# Autodesk Inventor assembly: am-3479L+6+SR+Mecanum+Left
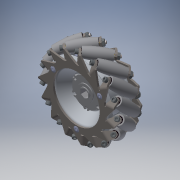
[picture p0: Inventor's stored thumbnail of the model, 180x180]
Saved by Autodesk Inventor 2016 SP2 (Build 200236200, 236)
## iProperties
Created: 2017-11-11
Part Number: am-3479L+6+SR+Mecanum+Left
Description: STEP AP214
Document SubType Name: Assembly
Designer: CAD
Sending System: SolidWorks 2017
Preprocessor: SwSTEP 2.0
Title: am-3479L 6 SR Mecanum Left.STEP
Revision Number: ANY
## Documents named in this file (8)
- C:\Users\CAD\Documents\GitHub\FIRST-ROBOTICS-2018-5436-CAD\Robot\Chassis\wheels\am-3479L+6+SR+Mecanum+Left.iam
- C:\Users\CAD\Documents\GitHub\FIRST-ROBOTICS-2018-5436-CAD\Robot\Chassis\wheels\ip-3479_hub.ipt
- C:\Users\CAD\Documents\GitHub\FIRST-ROBOTICS-2018-5436-CAD\Robot\Chassis\wheels\am-0676a Left Plate HD.ipt
- C:\Users\CAD\Documents\GitHub\FIRST-ROBOTICS-2018-5436-CAD\Robot\Chassis\wheels\am-3479_roller.iam
- C:\Users\CAD\Documents\GitHub\FIRST-ROBOTICS-2018-5436-CAD\Robot\Chassis\wheels\10-32x2250_shcs_HX-SHCS 0.19-32x1.375x1-C.ipt
- C:\Users\CAD\Documents\GitHub\FIRST-ROBOTICS-2018-5436-CAD\Robot\Chassis\wheels\10-32 Nylock Jam Nut_90633A411.ipt
- C:\Users\CAD\Documents\GitHub\FIRST-ROBOTICS-2018-5436-CAD\Robot\Chassis\wheels\am-1226 steel rivet 1875 125-250 grip.ipt
- C:\Users\CAD\Documents\GitHub\FIRST-ROBOTICS-2018-5436-CAD\Robot\Chassis\wheels\am-2568 500EX Hex Hub.ipt
## Components (56 placed, 56 different names)
1. ip-3479_hub_1 — Mate:1, Tangent:1, Tangent:2
2. ip-3479_hub_2
3. am-0676a Left Plate HD_3
4. am-0676a Left Plate HD_4
5. am-3479_roller_5 [sub-assembly]
6. 10-32x2250_shcs_HX-SHCS 0.19-32x1.375x1-C_6
7. 10-32 Nylock Jam Nut_90633A411_7
8. 10-32 Nylock Jam Nut_90633A411_8
9. 10-32 Nylock Jam Nut_90633A411_9
10. 10-32 Nylock Jam Nut_90633A411_10
11. 10-32 Nylock Jam Nut_90633A411_11
12. 10-32 Nylock Jam Nut_90633A411_12
13. 10-32 Nylock Jam Nut_90633A411_13
14. 10-32 Nylock Jam Nut_90633A411_14
15. 10-32 Nylock Jam Nut_90633A411_15
16. 10-32 Nylock Jam Nut_90633A411_16
17. 10-32 Nylock Jam Nut_90633A411_17
18. 10-32 Nylock Jam Nut_90633A411_18
19. 10-32 Nylock Jam Nut_90633A411_19
20. 10-32 Nylock Jam Nut_90633A411_20
21. 10-32 Nylock Jam Nut_90633A411_21
22. 10-32x2250_shcs_HX-SHCS 0.19-32x1.375x1-C_22
23. 10-32x2250_shcs_HX-SHCS 0.19-32x1.375x1-C_23
24. 10-32x2250_shcs_HX-SHCS 0.19-32x1.375x1-C_24
25. 10-32x2250_shcs_HX-SHCS 0.19-32x1.375x1-C_25
26. 10-32x2250_shcs_HX-SHCS 0.19-32x1.375x1-C_26
27. 10-32x2250_shcs_HX-SHCS 0.19-32x1.375x1-C_27
28. 10-32x2250_shcs_HX-SHCS 0.19-32x1.375x1-C_28
29. 10-32x2250_shcs_HX-SHCS 0.19-32x1.375x1-C_29
30. 10-32x2250_shcs_HX-SHCS 0.19-32x1.375x1-C_30
31. 10-32x2250_shcs_HX-SHCS 0.19-32x1.375x1-C_31
32. 10-32x2250_shcs_HX-SHCS 0.19-32x1.375x1-C_32
33. 10-32x2250_shcs_HX-SHCS 0.19-32x1.375x1-C_33
34. 10-32x2250_shcs_HX-SHCS 0.19-32x1.375x1-C_34
35. 10-32x2250_shcs_HX-SHCS 0.19-32x1.375x1-C_35
36. am-3479_roller_36 [sub-assembly]
37. am-3479_roller_37 [sub-assembly]
38. am-3479_roller_38 [sub-assembly]
39. am-3479_roller_39 [sub-assembly]
40. am-3479_roller_40 [sub-assembly]
41. am-3479_roller_41 [sub-assembly]
42. am-3479_roller_42 [sub-assembly]
43. am-3479_roller_43 [sub-assembly]
44. am-3479_roller_44 [sub-assembly]
45. am-3479_roller_45 [sub-assembly]
46. am-3479_roller_46 [sub-assembly]
47. am-3479_roller_47 [sub-assembly]
48. am-3479_roller_48 [sub-assembly]
49. am-3479_roller_49 [sub-assembly]
50. am-1226 steel rivet 1875 125-250 grip_50
51. am-1226 steel rivet 1875 125-250 grip_51
52. am-1226 steel rivet 1875 125-250 grip_52
53. am-1226 steel rivet 1875 125-250 grip_53
54. am-1226 steel rivet 1875 125-250 grip_54
55. am-1226 steel rivet 1875 125-250 grip_55
56. am-2568 500EX Hex Hub:1 — Mate:1, Tangent:1, Tangent:2
## Relationships (3: Tangent 2, Mate 1)
- Mate:1: ip-3479_hub_1 ↔ am-2568 500EX Hex Hub:1
- Tangent:1: ip-3479_hub_1 ↔ am-2568 500EX Hex Hub:1
- Tangent:2: ip-3479_hub_1 ↔ am-2568 500EX Hex Hub:1
